# Autodesk Inventor assembly: Motor Driver
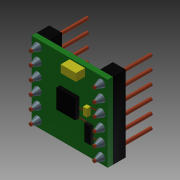
[picture p0: Inventor's stored thumbnail of the model, 180x180]
Saved by Autodesk Inventor 2013 (Build 170138000, 138)
## iProperties
Created: 2013-07-31
Part Number: Motor Driver
Document SubType Name: Assembly
Designer: Kyle
Author: Kyle
## Documents named in this file (9)
- C:\Users\Kyle\Documents\Inventor\2013\ROV\Motor Driver\Motor Driver.iam
- C:\Users\Kyle\Documents\Inventor\2013\ROV\Motor Driver\Board.ipt
- C:\Users\Kyle\Documents\Inventor\2013\ROV\Motor Driver\IC.ipt
- C:\Users\Kyle\Documents\Inventor\2013\ROV\Motor Driver\SMD Resistor LG.ipt
- C:\Users\Kyle\Documents\Inventor\2013\ROV\Motor Driver\SMD Resistor MD.ipt
- C:\Users\Kyle\Documents\Inventor\2013\ROV\Motor Driver\SMD Resistor SM.ipt
- C:\Users\Kyle\Documents\Inventor\2013\ROV\Motor Driver\PCB Wire SM.ipt
- C:\Users\Kyle\Documents\Inventor\2013\ROV\Motor Driver\Header.iam
- C:\Users\Kyle\Documents\Inventor\2013\ROV\Motor Driver\Solder Joint.ipt
## Components (23 placed, 8 different names)
1. Board:1 — Mate:1, Flush:1, Flush:2, Mate:2, Flush:3, Flush:4, Mate:3, Mate:4, Flush:7, Mate:5, Mate:8, Mate:11, Mate:12, Mate:13, Mate:14, Mate:15, Mate:16, Mate:23, Mate:24, Mate:25, Mate:26, Mate:27, Mate:28, Mate:29, Flush:11, Mate:31, Flush:12, Mate:39, Mate:40, Mate:41, Mate:42, Mate:43, Mate:44
2. IC:1 — Mate:1, Flush:1, Flush:2, Mate:6, Mate:9, Flush:9
3. SMD Resistor LG:1 — Mate:2, Flush:3, Flush:4
4. SMD Resistor MD:1 — Mate:3, Flush:10, Mate:10, Mate:32
5. SMD Resistor SM:1 — Mate:4, Flush:7, Flush:8, Mate:7, Mate:30
6. PCB Wire SM:1 — Mate:5, Mate:6, Flush:8, Mate:7
7. PCB Wire SM:2 — Mate:8, Mate:9, Flush:9, Flush:10, Mate:10
8. Header:1 [sub-assembly] — Mate:11, Mate:12, Mate:13, Mate:17, Mate:18, Mate:19, Mate:20, Mate:21, Mate:22
9. Header:2 [sub-assembly] — Mate:14, Mate:15, Mate:16, Mate:33, Mate:34, Mate:35, Mate:36, Mate:37, Mate:38
10. Solder Joint:1 — Mate:17, Mate:23
11. Solder Joint:2 — Mate:18, Mate:24
12. Solder Joint:3 — Mate:19, Mate:25
13. Solder Joint:4 — Mate:20, Mate:26
14. Solder Joint:5 — Mate:21, Mate:27
15. Solder Joint:6 — Mate:22, Mate:28
16. PCB Wire SM:3 — Mate:31, Mate:32, Flush:12
17. PCB Wire SM:4 — Mate:29, Mate:30, Flush:11
18. Solder Joint:7 — Mate:38, Mate:44
19. Solder Joint:8 — Mate:37, Mate:43
20. Solder Joint:9 — Mate:36, Mate:42
21. Solder Joint:10 — Mate:35, Mate:41
22. Solder Joint:11 — Mate:34, Mate:40
23. Solder Joint:12 — Mate:33, Mate:39
## Relationships (54: Mate 44, Flush 10)
- Mate:1: Board:1 ↔ IC:1
- Flush:1 (5.715 mm): Board:1 ↔ IC:1
- Flush:2 (5.715 mm): Board:1 ↔ IC:1
- Mate:2: Board:1 ↔ SMD Resistor LG:1
- Flush:3 (0.254 mm): Board:1 ↔ SMD Resistor LG:1
- Flush:4 (4.572 mm): Board:1 ↔ SMD Resistor LG:1
- Mate:3: Board:1 ↔ SMD Resistor MD:1
- Mate:4: Board:1 ↔ SMD Resistor SM:1
- Flush:7 (6.35 mm): Board:1 ↔ SMD Resistor SM:1
- Mate:5: Board:1 ↔ PCB Wire SM:1
- Mate:6: IC:1 ↔ PCB Wire SM:1
- Flush:8: SMD Resistor SM:1 ↔ PCB Wire SM:1
- Mate:7: SMD Resistor SM:1 ↔ PCB Wire SM:1
- Mate:8: Board:1 ↔ PCB Wire SM:2
- Mate:9: IC:1 ↔ PCB Wire SM:2
- Flush:9: IC:1 ↔ PCB Wire SM:2
- Flush:10: SMD Resistor MD:1 ↔ PCB Wire SM:2
- Mate:10: SMD Resistor MD:1 ↔ PCB Wire SM:2
- Mate:11: Board:1 ↔ Header:1
- Mate:12: Board:1 ↔ Header:1
- Mate:13: Board:1 ↔ Header:1
- Mate:14: Board:1 ↔ Header:2
- Mate:15: Board:1 ↔ Header:2
- Mate:16: Board:1 ↔ Header:2
- Mate:17: Header:1 ↔ Solder Joint:1
- Mate:18: Header:1 ↔ Solder Joint:2
- Mate:19: Header:1 ↔ Solder Joint:3
- Mate:20: Header:1 ↔ Solder Joint:4
- Mate:21: Header:1 ↔ Solder Joint:5
- Mate:22: Header:1 ↔ Solder Joint:6
- Mate:23: Board:1 ↔ Solder Joint:1
- Mate:24: Board:1 ↔ Solder Joint:2
- Mate:25: Board:1 ↔ Solder Joint:3
- Mate:26: Board:1 ↔ Solder Joint:4
- Mate:27: Board:1 ↔ Solder Joint:5
- Mate:28: Board:1 ↔ Solder Joint:6
- Mate:29: Board:1 ↔ PCB Wire SM:4
- Mate:30: SMD Resistor SM:1 ↔ PCB Wire SM:4
- Flush:11 (8.636 mm): Board:1 ↔ PCB Wire SM:4
- Mate:31: Board:1 ↔ PCB Wire SM:3
- Mate:32: SMD Resistor MD:1 ↔ PCB Wire SM:3
- Flush:12 (3.556 mm): Board:1 ↔ PCB Wire SM:3
- Mate:33: Header:2 ↔ Solder Joint:12
- Mate:34: Header:2 ↔ Solder Joint:11
- Mate:35: Header:2 ↔ Solder Joint:10
- Mate:36: Header:2 ↔ Solder Joint:9
- Mate:37: Header:2 ↔ Solder Joint:8
- Mate:38: Header:2 ↔ Solder Joint:7
- Mate:39: Board:1 ↔ Solder Joint:12
- Mate:40: Board:1 ↔ Solder Joint:11
- Mate:41: Board:1 ↔ Solder Joint:10
- Mate:42: Board:1 ↔ Solder Joint:9
- Mate:43: Board:1 ↔ Solder Joint:8
- Mate:44: Board:1 ↔ Solder Joint:7
